# Autodesk Inventor assembly: Assembly tarea
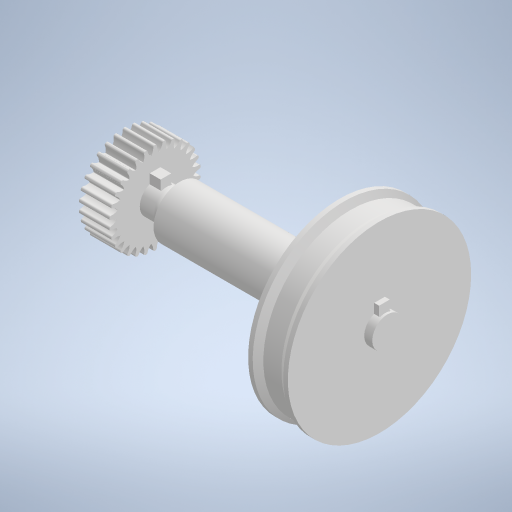
[picture p0: Inventor's stored thumbnail of the model, 512x512]
Saved by Autodesk Inventor 2023 (Build 270158000, 158)
## iProperties
Created: 2024-03-27
Part Number: Assembly tarea
Document SubType Name: Assembly
Designer: kikev
Author: kikev
## Documents named in this file (5)
- C:\Users\kikev\OneDrive - Universidad Rafael Landivar\Documentos\SEMESTRE VII\DINAMICA\Assembly tarea.iam
- C:\Users\kikev\OneDrive - Universidad Rafael Landivar\Documentos\SEMESTRE VII\DINAMICA\Cuña.ipt
- C:\Users\kikev\OneDrive - Universidad Rafael Landivar\Documentos\SEMESTRE VII\DINAMICA\EJE_CUÑEROS (1).ipt
- C:\Users\kikev\OneDrive - Universidad Rafael Landivar\Documentos\SEMESTRE VII\DINAMICA\POLEA.ipt
- C:\Users\kikev\OneDrive - Universidad Rafael Landivar\Documentos\SEMESTRE VII\DINAMICA\ENGRANE.ipt
## Components (5 placed, 4 different names)
1. Cuña:1 — Planar:1
2. EJE_CUÑEROS (1):1 — Mate:1, Planar:1, Rigid:1, Planar:2
3. POLEA:1 — Mate:1
4. ENGRANE:1 — Rigid:1
5. Cuña:2 — Planar:2
## Relationships (4: PlanarJoint 2, Mate 1, WeldJoint 1)
- Mate:1: EJE_CUÑEROS (1):1 ↔ POLEA:1
- Planar:1: Cuña:1 ↔ EJE_CUÑEROS (1):1
- Rigid:1 [WeldJoint]: EJE_CUÑEROS (1):1 ↔ ENGRANE:1
- Planar:2: EJE_CUÑEROS (1):1 ↔ Cuña:2
